# Autodesk Inventor assembly: Assembly
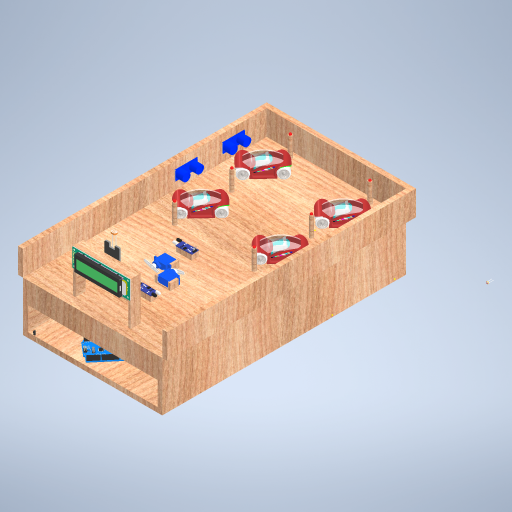
[picture p0: Inventor's stored thumbnail of the model, 512x512]
Saved by Autodesk Inventor 2024.3 (Build 283343000, 343)
## iProperties
Created: 2024-12-06
Part Number: Assembly
Document SubType Name: Assembly
Designer: PRE 7730
Author: PRE 7730
## Documents named in this file (13)
- A:\ASU\senior 1\semster 1\Sensors and Measurement Systems\Project\inventor\Assembly.iam
- A:\ASU\senior 1\semster 1\Sensors and Measurement Systems\Project\SOLID\hw-201-ir-infrared-obstacle-avoidance-sensor-1.snapshot.24\Infrared Obstacle Detecting Module v4\Infrared Obstacle Detecting Module v4\Inf.ipt
- A:\ASU\senior 1\semster 1\Sensors and Measurement Systems\Project\SOLID\hc-sr04-ultrasonic-sensor-11.snapshot.1\ultrasonik_sensor_\ultrasonik_sensor_\ultrasonik_sensor_.ipt
- A:\ASU\senior 1\semster 1\Sensors and Measurement Systems\Project\SOLID\lm-35-1.snapshot.2\lm35\lm35\lm35.ipt
- A:\ASU\senior 1\semster 1\Sensors and Measurement Systems\Project\SOLID\ldr-5mm-1.snapshot.1\LDR v1\LDR v1\LDR v1.ipt
- A:\ASU\senior 1\semster 1\Sensors and Measurement Systems\Project\SOLID\servo-motor-112.snapshot.1\Servo motor\Servo motor\Servo motor.ipt
- A:\ASU\senior 1\semster 1\Sensors and Measurement Systems\Project\inventor\box.ipt
- A:\ASU\senior 1\semster 1\Sensors and Measurement Systems\Project\SOLID\Car\Car\Car.ipt
- A:\ASU\senior 1\semster 1\Sensors and Measurement Systems\Project\SOLID\ERM2002-1\ERM2002-1\ERM2002-1.ipt
- A:\ASU\senior 1\semster 1\Sensors and Measurement Systems\Project\SOLID\freshly-squeezed-1.snapshot.7\Assembly\Assembly\Assembly.ipt
- A:\ASU\senior 1\semster 1\Sensors and Measurement Systems\Project\SOLID\5mm-led-red-1.snapshot.1\LED5mm\LED5mm\LED5mm.ipt
- A:\ASU\senior 1\semster 1\Sensors and Measurement Systems\Project\SOLID\LDR\LDR\LDR.ipt
- A:\ASU\senior 1\semster 1\Sensors and Measurement Systems\Project\SOLID\arduinoUnoCH340_USB-B_v2\arduinoUnoCH340_USB-B_v2\arduinoUnoCH340_USB-B_v2.ipt
## Components (25 placed, 12 different names)
1. Inf:1 — Mate:2, Mate:3
2. Inf:2 — Mate:4, Mate:5
3. ultrasonik_sensor_:1 — Mate:12, Mate:13, Mate:14
4. ultrasonik_sensor_:2 — Mate:25, Mate:26
5. ultrasonik_sensor_:3 — Mate:23, Mate:24
6. ultrasonik_sensor_:4 — Mate:15, Mate:16, Mate:17
7. lm35:1 — Mate:50
8. LDR v1:1
9. box:1 — Mate:1, Mate:2, Mate:3, Mate:4, Mate:5, Mate:12, Mate:13, Mate:14, Mate:15, Mate:16, Mate:17, Mate:23, Mate:24, Mate:25, Mate:26, Mate:27, Mate:28, Mate:29, Mate:30, Mate:31, Mate:32, Mate:33, Mate:34, Mate:35, Mate:36, Mate:37, Mate:38, Mate:39, Mate:40, Mate:41, Mate:42, Mate:43, Mate:44, Mate:45, Mate:46, Mate:47, Mate:48, Mate:49, Mate:50
10. Car:1 — Mate:28
11. ERM2002-1:1 — Mate:1, Mate:37, Mate:38, Mate:39
12. Car:2 — Mate:29
13. Car:3 — Mate:27
14. Car:4 — Mate:30
15. Servo motor:2 — Mate:31, Mate:32, Mate:33
16. Servo motor:3 — Mate:34, Mate:35, Mate:36
17. Assembly:1
18. LED5mm:1 — Mate:42
19. LED5mm:2 — Mate:41
20. LED5mm:3 — Mate:40
21. LED5mm:4 — Mate:44
22. LED5mm:5 — Mate:43
23. LED5mm:6 — Mate:45
24. LDR:1 — Mate:46, Mate:47, Mate:48
25. arduinoUnoCH340_USB-B_v2:1 — Mate:49
## Relationships (39: Mate 39)
- Mate:1: box:1 ↔ ERM2002-1:1
- Mate:2: Inf:1 ↔ box:1
- Mate:3: Inf:1 ↔ box:1
- Mate:4: Inf:2 ↔ box:1
- Mate:5: Inf:2 ↔ box:1
- Mate:12: ultrasonik_sensor_:1 ↔ box:1
- Mate:13: ultrasonik_sensor_:1 ↔ box:1
- Mate:14: ultrasonik_sensor_:1 ↔ box:1
- Mate:15: ultrasonik_sensor_:4 ↔ box:1
- Mate:16: ultrasonik_sensor_:4 ↔ box:1
- Mate:17: ultrasonik_sensor_:4 ↔ box:1
- Mate:23: ultrasonik_sensor_:3 ↔ box:1
- Mate:24: ultrasonik_sensor_:3 ↔ box:1
- Mate:25: ultrasonik_sensor_:2 ↔ box:1
- Mate:26: ultrasonik_sensor_:2 ↔ box:1
- Mate:27: box:1 ↔ Car:3
- Mate:28: box:1 ↔ Car:1
- Mate:29: box:1 ↔ Car:2
- Mate:30: box:1 ↔ Car:4
- Mate:31: box:1 ↔ Servo motor:2
- Mate:32: box:1 ↔ Servo motor:2
- Mate:33: box:1 ↔ Servo motor:2
- Mate:34: box:1 ↔ Servo motor:3
- Mate:35: box:1 ↔ Servo motor:3
- Mate:36: box:1 ↔ Servo motor:3
- Mate:37: box:1 ↔ ERM2002-1:1
- Mate:38: box:1 ↔ ERM2002-1:1
- Mate:39: box:1 ↔ ERM2002-1:1
- Mate:40: box:1 ↔ LED5mm:3
- Mate:41: box:1 ↔ LED5mm:2
- Mate:42: box:1 ↔ LED5mm:1
- Mate:43: box:1 ↔ LED5mm:5
- Mate:44: box:1 ↔ LED5mm:4
- Mate:45: box:1 ↔ LED5mm:6
- Mate:46: box:1 ↔ LDR:1
- Mate:47: box:1 ↔ LDR:1
- Mate:48: box:1 ↔ LDR:1
- Mate:49: box:1 ↔ arduinoUnoCH340_USB-B_v2:1
- Mate:50: lm35:1 ↔ box:1
